# Autodesk Inventor assembly: Encoder_Mount1
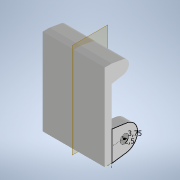
[picture p0: Inventor's stored thumbnail of the model, 180x180]
Saved by Autodesk Inventor 2022 (Build 260153000, 153)
## iProperties
Created: 2024-04-26
Part Number: Encoder_Mount1
Document SubType Name: Assembly
Designer: raphael.hauk
Author: raphael.hauk
## Documents named in this file (3)
- C:\git\inkjet-printer\cad\Encoder_Mount1.iam
- C:\git\inkjet-printer\cad\Enoder_Mount1.ipt
- C:\git\inkjet-printer\cad\Encoder_Mount1_Slider.ipt
## Components (2 placed, 2 different names)
1. Enoder_Mount1:1 — Flush:1
2. Encoder_Mount1_Slider:1 — Flush:1
## Relationships (1: Flush 1)
- Flush:1: Enoder_Mount1:1 ↔ Encoder_Mount1_Slider:1
